# Autodesk Inventor assembly: final2
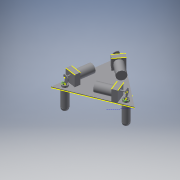
[picture p0: Inventor's stored thumbnail of the model, 180x180]
Saved by Autodesk Inventor 2018 (Build 220112000, 112)
## iProperties
Created: 2019-05-30
Part Number: final2
Document SubType Name: Assembly
Designer: DELL
Author: DELL
## Documents named in this file (6)
- C:\Users\DELL\Downloads\final2.iam
- C:\Users\DELL\Downloads\motor2.iam
- C:\Users\DELL\Downloads\base1.ipt
- C:\Users\DELL\Downloads\Assembly2.iam
- C:\Users\DELL\Downloads\guide1.ipt
- C:\Users\DELL\Downloads\pusher.ipt
## Components (13 placed, 5 different names)
1. motor2:1 [sub-assembly] — Mate:4, Flush:1, Mate:5
2. motor2:2 [sub-assembly] — Mate:6, Flush:2, Mate:7
3. motor2:3 [sub-assembly] — Mate:8, Flush:3, Mate:9
4. base1:1 — Rotational:1, Rotational:2, Rotational:3, Rotational:4, Rotational:5, Rotational:6, Mate:4, Flush:1, Mate:6, Flush:2, Mate:8, Flush:3
5. Assembly2:1 [sub-assembly] — Rotational:4, Mate:3
6. Assembly2:2 [sub-assembly] — Rotational:5, Mate:2
7. Assembly2:3 [sub-assembly] — Rotational:6
8. guide1:1 — Rotational:1, Mate:1
9. guide1:2 — Rotational:2
10. guide1:3 — Rotational:3
11. pusher:1 — Mate:3, Mate:7
12. pusher:2 — Mate:2, Mate:5
13. pusher:3 — Mate:1, Mate:9
## Relationships (18: Mate 9, RevoluteJoint 6, Flush 3)
- Rotational:1 [RevoluteJoint]: base1:1 ↔ guide1:1
- Rotational:2 [RevoluteJoint]: base1:1 ↔ guide1:2
- Rotational:3 [RevoluteJoint]: base1:1 ↔ guide1:3
- Rotational:4 [RevoluteJoint]: base1:1 ↔ Assembly2:1
- Rotational:5 [RevoluteJoint]: base1:1 ↔ Assembly2:2
- Rotational:6 [RevoluteJoint]: base1:1 ↔ Assembly2:3
- Mate:1: guide1:1 ↔ pusher:3
- Mate:2: Assembly2:2 ↔ pusher:2
- Mate:3: Assembly2:1 ↔ pusher:1
- Mate:4: motor2:1 ↔ base1:1
- Flush:1: motor2:1 ↔ base1:1
- Mate:5: motor2:1 ↔ pusher:2
- Mate:6: motor2:2 ↔ base1:1
- Flush:2: motor2:2 ↔ base1:1
- Mate:7: motor2:2 ↔ pusher:1
- Mate:8: motor2:3 ↔ base1:1
- Flush:3: motor2:3 ↔ base1:1
- Mate:9: motor2:3 ↔ pusher:3
